# Autodesk Inventor assembly: MotorEncoderAssembly
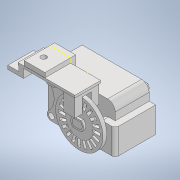
[picture p0: Inventor's stored thumbnail of the model, 180x180]
Saved by Autodesk Inventor 2022 (Build 260153070, 153G)
## iProperties
Created: 2021-11-27
Part Number: MotorEncoderAssembly
Document SubType Name: Assembly
Designer: a laptop
Author: a laptop
## Documents named in this file (5)
- C:\Users\a laptop\Desktop\SumoBot\sumobotENCODER\MotorEncoderAssembly.iam
- C:\Users\a laptop\Desktop\SumoBot\sumobotENCODER\LM393 encoder.ipt
- C:\Users\a laptop\Desktop\SumoBot\sumobotENCODER\TT encoder disk.ipt
- C:\Users\a laptop\Desktop\SumoBot\sumobotENCODER\TT motor output.ipt
- C:\Users\a laptop\Desktop\SumoBot\sumobotENCODER\MotorEncoderBracket.ipt
## Components (4 placed, 4 different names)
1. LM393 encoder:1 — Angle:2, Angle:3, Mate:3, Mate:8, Tangent:1
2. TT encoder disk:1 — Mate:1, Angle:1, Flush:1, Mate:2, Mate:3, Tangent:1
3. TT motor output:1 — Mate:1, Angle:1, Flush:1, Mate:2, Angle:2, Angle:3, Mate:4, Mate:5, Flush:2
4. MotorEncoderBracket:1 — Flush:2
## Relationships (15: Mate 9, Angle 3, Flush 2, Tangent 1)
- Mate:1: TT encoder disk:1 ↔ TT motor output:1
- Angle:1 (0 deg): TT encoder disk:1 ↔ TT motor output:1
- Flush:1: TT encoder disk:1 ↔ TT motor output:1
- Mate:2: TT encoder disk:1 ↔ TT motor output:1
- Angle:2 (180 deg): LM393 encoder:1 ↔ TT motor output:1
- Angle:3 (180 deg): LM393 encoder:1 ↔ TT motor output:1
- Mate:3 (1.5 mm): LM393 encoder:1 ↔ TT encoder disk:1
- Mate:4: TT motor output:1
- Mate:5: TT motor output:1
- Mate:6
- Mate:7
- Mate:8: LM393 encoder:1
- Mate:9 (0.925 mm)
- Tangent:1 (1.5 mm): LM393 encoder:1 ↔ TT encoder disk:1
- Flush:2: TT motor output:1 ↔ MotorEncoderBracket:1
